# Autodesk Inventor assembly: Omni Wheel No Shaft
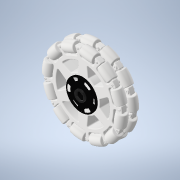
[picture p0: Inventor's stored thumbnail of the model, 180x180]
Saved by Autodesk Inventor 2020 (Build 240168000, 168)
## iProperties
Created: 2020-01-25
Part Number: Omni Wheel No Shaft
Document SubType Name: Assembly
Designer: aidan
Author: aidan
## Documents named in this file (4)
- C:\Users\aidan\Desktop\T3 Robotics\CAD\Omni Wheel No Shaft.iam
- C:\Users\aidan\Desktop\T3 Robotics\CAD\0.5in Hex Hub.ipt
- C:\Users\aidan\Desktop\T3 Robotics\CAD\STEP Files\6_Omni-Directional_Wheel_217-2585.ipt
- C:\Users\aidan\Desktop\T3 Robotics\CAD\Generic and Stock\Hex Spacer STOCK.ipt
## Components (4 placed, 3 different names)
1. 0.5in Hex Hub:1 — Mate:1, Mate:2, Mate:6, Mate:7, Flush:10
2. 0.5in Hex Hub:2 — Mate:3, Mate:4, Mate:5, Flush:9
3. 6_Omni-Directional_Wheel_217-2585:1 — Mate:1, Mate:2, Mate:3, Mate:4, Mate:5, Mate:6
4. Hex Spacer STOCK:1 — Mate:7, Flush:9, Flush:10
## Relationships (9: Mate 7, Flush 2)
- Mate:1: 0.5in Hex Hub:1 ↔ 6_Omni-Directional_Wheel_217-2585:1
- Mate:2: 0.5in Hex Hub:1 ↔ 6_Omni-Directional_Wheel_217-2585:1
- Mate:3: 0.5in Hex Hub:2 ↔ 6_Omni-Directional_Wheel_217-2585:1
- Mate:4: 0.5in Hex Hub:2 ↔ 6_Omni-Directional_Wheel_217-2585:1
- Mate:5: 0.5in Hex Hub:2 ↔ 6_Omni-Directional_Wheel_217-2585:1
- Mate:6: 0.5in Hex Hub:1 ↔ 6_Omni-Directional_Wheel_217-2585:1
- Mate:7: 0.5in Hex Hub:1 ↔ Hex Spacer STOCK:1
- Flush:9: 0.5in Hex Hub:2 ↔ Hex Spacer STOCK:1
- Flush:10: 0.5in Hex Hub:1 ↔ Hex Spacer STOCK:1
